# Autodesk Inventor assembly: rev3
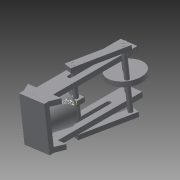
[picture p0: Inventor's stored thumbnail of the model, 180x180]
Saved by Autodesk Inventor 2015 (Build 190159000, 159)
## iProperties
Created: 2014-07-15
Part Number: rev3
Document SubType Name: Assembly
Designer: shohei
Author: shohei
## Documents named in this file (10)
- C:\Users\shohei\Documents\Inventor\FufuPounder\rev3.iam
- C:\Users\shohei\Documents\Inventor\FufuPounder\mortar.ipt
- C:\Users\shohei\Documents\Inventor\FufuPounder\Part1.ipt
- C:\Users\shohei\Documents\Inventor\FufuPounder\Part2.ipt
- C:\Users\shohei\Documents\Inventor\FufuPounder\pulley.ipt
- C:\Users\shohei\Documents\Inventor\FufuPounder\Part4.ipt
- C:\Users\shohei\Documents\Inventor\FufuPounder\baseboard.ipt
- C:\Users\shohei\Documents\Inventor\FufuPounder\shaft2.ipt
- C:\Users\shohei\Documents\Inventor\FufuPounder\shaft3.ipt
- C:\Users\shohei\Documents\Inventor\FufuPounder\mallet_aseembly.iam
## Components (11 placed, 9 different names)
1. mortar:1 — Mate:1
2. Part1:1 — Flush:3, Rigid:2, Mate:4, Flush:5
3. Part1:2 — Flush:3, Mate:2, Mate:3, Flush:4, Mate:5, Slider:1
4. pulley:1 — Cylindrical:11, Cylindrical:12, Angle:1
5. Part4:1 — Rotational:4, Rotational:6
6. Part4:2 — Rotational:5, Rotational:7
7. Part2:3 — Rigid:2, Cylindrical:11
8. baseboard:1 — Mate:2, Mate:3, Mate:4, Flush:4, Mate:5, Flush:5, Angle:1
9. shaft2:1 — Cylindrical:14, Slider:1, Rotational:6, Rotational:7
10. shaft3:1 — Rotational:4, Rotational:5, Cylindrical:12
11. mallet_aseembly:1 [sub-assembly] — Cylindrical:14
## Relationships (18: Mate 5, RevoluteJoint 4, Flush 3, CylindricalJoint 3, WeldJoint 1, Angle 1, TranslationJoint 1)
- Mate:1: mortar:1
- Flush:3: Part1:1 ↔ Part1:2
- Rigid:2 [WeldJoint]: Part1:1 ↔ Part2:3
- Cylindrical:11: pulley:1 ↔ Part2:3
- Mate:2: Part1:2 ↔ baseboard:1
- Mate:3: Part1:2 ↔ baseboard:1
- Mate:4: Part1:1 ↔ baseboard:1
- Flush:4: Part1:2 ↔ baseboard:1
- Mate:5: Part1:2 ↔ baseboard:1
- Flush:5: Part1:1 ↔ baseboard:1
- Rotational:4 [RevoluteJoint]: Part4:1 ↔ shaft3:1
- Rotational:5 [RevoluteJoint]: Part4:2 ↔ shaft3:1
- Cylindrical:12: pulley:1 ↔ shaft3:1
- Cylindrical:14: shaft2:1 ↔ mallet_aseembly:1
- Angle:1 (2000 deg): pulley:1 ↔ baseboard:1
- Slider:1 [TranslationJoint] (-10 mm): Part1:2 ↔ shaft2:1
- Rotational:6 [RevoluteJoint]: Part4:1 ↔ shaft2:1
- Rotational:7 [RevoluteJoint]: Part4:2 ↔ shaft2:1
